# Autodesk Inventor assembly: Storage System Assembly
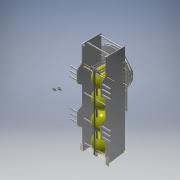
[picture p0: Inventor's stored thumbnail of the model, 180x180]
Saved by Autodesk Inventor 2019.4 (Build 234330000, 330)
## iProperties
Created: 2020-01-24
Part Number: Storage System Assembly
Document SubType Name: Assembly
Designer: admin
Mass: 6812.94 g
Surface Area: 16983.8 cm^2
Volume: 14320.1 cm^3
Density: 0.47576 g/cm^3
Author: admin
## Documents named in this file (18)
- C:\Users\admin\Desktop\FRC 2020 Engineering\GitHub\7738-2020\Robot V2\Storage System\Storage System Assembly.iam
- C:\Users\admin\Desktop\FRC 2020 Engineering\GitHub\7738-2020\Robot V2\Storage System\Storage Side Plate.ipt
- C:\Users\admin\Desktop\FRC 2020 Engineering\GitHub\7738-2020\Robot V2\Storage System\Storage System Assembly\Design Accelerator\Synchronous Belts Transmission1.iam
- C:\Users\admin\Desktop\FRC 2020 Engineering\GitHub\7738-2020\Robot V2\Storage System\Storage System Assembly\Design Accelerator\Synchronous Belts Transmission3.iam
- C:\Users\admin\Desktop\FRC 2020 Engineering\GitHub\7738-2020\Robot V2\Storage System\Storage System Assembly\Design Accelerator\Synchronous Belts Transmission4.iam
- C:\Users\admin\Desktop\FRC 2020 Engineering\GitHub\7738-2020\Robot V2\Storage System\Storage System Assembly\Design Accelerator\Synchronous Belts Transmission5.iam
- C:\Users\admin\Desktop\FRC 2020 Engineering\GitHub\7738-2020\Robot V2\Storage System\Storage System Assembly\Design Accelerator\Synchronous Belts Transmission6.iam
- C:\Users\admin\Desktop\FRC 2020 Engineering\GitHub\7738-2020\Power Cell.ipt
- C:\Users\admin\Desktop\FRC 2020 Engineering\GitHub\7738-2020\Robot V2\Turret\F6800.ipt
- C:\Users\admin\Desktop\FRC 2020 Engineering\GitHub\7738-2020\Robot V2\Storage System\Turret Support 2.ipt
- C:\Users\admin\Desktop\FRC 2020 Engineering\GitHub\7738-2020\Robot V2\Storage System\Turret Support.ipt
- C:\Users\admin\Desktop\FRC 2020 Engineering\GitHub\7738-2020\Robot V2\Storage System\Mounting Bracket.ipt
- C:\Users\admin\Desktop\FRC 2020 Engineering\GitHub\7738-2020\Robot V2\Storage System\Mounting Bracket 2.ipt
- C:\Users\admin\Desktop\FRC 2020 Engineering\GitHub\7738-2020\Robot V2\Storage System\Storage Plate Spacer.ipt
- C:\Users\admin\Desktop\FRC 2020 Engineering\GitHub\7738-2020\Robot V2\Storage System\Turret Bracket.ipt
- C:\Users\admin\Desktop\FRC 2020 Engineering\GitHub\7738-2020\Robot V2\Storage System\Small Support.ipt
- C:\Users\admin\Desktop\FRC 2020 Engineering\GitHub\7738-2020\Robot V2\Turret\Storage mounting spacers.ipt
- C:\Users\admin\Desktop\FRC 2020 Engineering\GitHub\7738-2020\Upper Stage\KFL08.ipt
## Components (61 placed, 13 different names)
1. Storage Side Plate:1 — Mate:1, Mate:3, Flush:2, Mate:14, Mate:15, Mate:16, Mate:17, Mate:25, Mate:26, Mate:27, Mate:28, Mate:31, Mate:32, Mate:38, Flush:3, Mate:43, Flush:7, Flush:8, Mate:44, Mate:45, Mate:46, Mate:47, Mate:48, Mate:49, Mate:50, Mate:51, Mate:52, Mate:63, Flush:13, Flush:15, Mate:92, Flush:17, Mate:94, Mate:108, Mate:109, Mate:110, Mate:111, Mate:112, Mate:113, Mate:114, Mate:115, Mate:116, Mate:117, Mate:118, Mate:119
2. Storage Side Plate:2 — Mate:1, Flush:1, Mate:12, Mate:13, Mate:18, Mate:19, Mate:20, Mate:22, Mate:23, Mate:24, Mate:29, Mate:30, Mate:40, Flush:4, Mate:42, Flush:5, Flush:6, Mate:53, Mate:54, Mate:55, Mate:56, Mate:57, Mate:58, Mate:59, Mate:60, Mate:61, Flush:9, Mate:65, Flush:11, Mate:80, Flush:14, Mate:126, Mate:127, Mate:128, Mate:129, Mate:130, Mate:131, Mate:132, Mate:133, Mate:134, Mate:135, Mate:136, Mate:137
3. Synchronous Belts Transmission:1 [sub-assembly]
4. Synchronous Belts Transmission:2 [sub-assembly]
5. Synchronous Belts Transmission:3 [sub-assembly]
6. Synchronous Belts Transmission:4 [sub-assembly]
7. Synchronous Belts Transmission:5 [sub-assembly]
8. Power Cell:1 — Mate:4, Mate:8
9. Power Cell:2 — Mate:5, Mate:11
10. Power Cell:3 — Mate:6, Mate:9
11. Power Cell:4 — Mate:7, Mate:10
12. F6800:1 — Mate:13, Mate:24
13. F6800:2 — Mate:30
14. F6800:3 — Mate:19, Mate:22
15. F6800:4 — Mate:14, Mate:25
16. F6800:5 — Mate:15, Mate:26
17. F6800:7 — Mate:16, Mate:28
18. F6800:8 — Mate:17, Mate:27
19. F6800:9 — Mate:18, Mate:29
20. F6800:10 — Mate:20, Mate:23
21. F6800:11 — Mate:31, Mate:32
22. Mounting Bracket:1 — Mate:38, Flush:3, Flush:13
23. Mounting Bracket:2 — Mate:40, Flush:4, Flush:14
24. Mounting Bracket 2:1 — Mate:42, Flush:5, Flush:6
25. Mounting Bracket 2:2 — Mate:43, Flush:7, Flush:8
26. Storage Plate Spacer:1 — Mate:46, Mate:60
27. Storage Plate Spacer:2 — Mate:48, Mate:55
28. Storage Plate Spacer:3 — Mate:44, Mate:59
29. Storage Plate Spacer:4 — Mate:51, Mate:54
30. Storage Plate Spacer:5 — Mate:47, Mate:80
31. Storage Plate Spacer:6 — Mate:50, Mate:57
32. Storage Plate Spacer:7 — Mate:49, Mate:56
33. Storage Plate Spacer:8 — Mate:52, Mate:53
34. Storage Plate Spacer:9 — Mate:45, Mate:58
35. Turret Bracket:2 — Mate:61, Flush:9, Flush:11
36. Turret Bracket:3 — Mate:65, Flush:16
37. Turret Bracket:4 — Mate:63, Flush:15, Flush:16, Mate:95
38. Small Support:1 — Mate:104, Mate:107
39. Small Support:2 — Mate:102, Mate:103
40. Small Support:3 — Mate:105, Mate:106
41. Small Support:4 — Mate:99, Mate:100, Mate:101
42. Turret Bracket:5 — Mate:92, Flush:17, Mate:98, Mate:100, Mate:103
43. Turret Support 2:2 — Mate:97, Mate:98, Mate:99, Mate:101, Mate:102, Mate:104, Mate:105, Mate:106, Mate:107
44. Turret Support:3 — Mate:93, Mate:94, Mate:95, Mate:96, Mate:97
45. Storage mounting spacers:1 — Mate:108, Mate:119
46. Storage mounting spacers:2 — Mate:109, Mate:118
47. Storage mounting spacers:3 — Mate:110, Mate:117
48. Storage mounting spacers:4 — Mate:111, Mate:114
49. Storage mounting spacers:5 — Mate:112, Mate:115
50. Storage mounting spacers:6 — Mate:113, Mate:116
51. Storage mounting spacers:7 — Mate:126, Mate:137
52. Storage mounting spacers:8 — Mate:127, Mate:136
53. Storage mounting spacers:9 — Mate:128, Mate:135
54. Storage mounting spacers:10 — Mate:130, Mate:133
55. Storage mounting spacers:11 — Mate:129, Mate:134
56. Storage mounting spacers:12 — Mate:131, Mate:132
57. KFL08:1
58. KFL08:2
59. KFL08:3
60. KFL08:4
61. KFL08:5
## Relationships (110: Mate 95, Flush 15)
- Mate:1: Storage Side Plate:1 ↔ Storage Side Plate:2
- Mate:3 (114.3 mm): Storage Side Plate:1
- Flush:1 (114.3 mm): Storage Side Plate:2
- Mate:4: Power Cell:1
- Mate:5: Power Cell:2
- Mate:6: Power Cell:3
- Mate:7: Power Cell:4
- Mate:8: Power Cell:1
- Mate:9: Power Cell:3
- Mate:10: Power Cell:4
- Mate:11: Power Cell:2
- Mate:12: Storage Side Plate:2
- Flush:2: Storage Side Plate:1
- Mate:13: Storage Side Plate:2 ↔ F6800:1
- Mate:14: Storage Side Plate:1 ↔ F6800:4
- Mate:15: Storage Side Plate:1 ↔ F6800:5
- Mate:16: Storage Side Plate:1 ↔ F6800:7
- Mate:17: Storage Side Plate:1 ↔ F6800:8
- Mate:18: Storage Side Plate:2 ↔ F6800:9
- Mate:19: Storage Side Plate:2 ↔ F6800:3
- Mate:20: Storage Side Plate:2 ↔ F6800:10
- Mate:22 (0.2 mm): Storage Side Plate:2 ↔ F6800:3
- Mate:23 (0.2 mm): Storage Side Plate:2 ↔ F6800:10
- Mate:24 (0.2 mm): Storage Side Plate:2 ↔ F6800:1
- Mate:25 (0.2 mm): Storage Side Plate:1 ↔ F6800:4
- Mate:26 (0.2 mm): Storage Side Plate:1 ↔ F6800:5
- Mate:27 (0.2 mm): Storage Side Plate:1 ↔ F6800:8
- Mate:28 (0.2 mm): Storage Side Plate:1 ↔ F6800:7
- Mate:29 (0.2 mm): Storage Side Plate:2 ↔ F6800:9
- Mate:30 (0.2 mm): Storage Side Plate:2 ↔ F6800:2
- Mate:31: Storage Side Plate:1 ↔ F6800:11
- Mate:32 (0.2 mm): Storage Side Plate:1 ↔ F6800:11
- Mate:38: Storage Side Plate:1 ↔ Mounting Bracket:1
- Flush:3 (5 mm): Storage Side Plate:1 ↔ Mounting Bracket:1
- Mate:40: Storage Side Plate:2 ↔ Mounting Bracket:2
- Flush:4 (5 mm): Storage Side Plate:2 ↔ Mounting Bracket:2
- Mate:42: Storage Side Plate:2 ↔ Mounting Bracket 2:1
- Mate:43: Storage Side Plate:1 ↔ Mounting Bracket 2:2
- Flush:5: Storage Side Plate:2 ↔ Mounting Bracket 2:1
- Flush:6: Storage Side Plate:2 ↔ Mounting Bracket 2:1
- Flush:7: Storage Side Plate:1 ↔ Mounting Bracket 2:2
- Flush:8: Storage Side Plate:1 ↔ Mounting Bracket 2:2
- Mate:44: Storage Side Plate:1 ↔ Storage Plate Spacer:3
- Mate:45: Storage Side Plate:1 ↔ Storage Plate Spacer:9
- Mate:46: Storage Side Plate:1 ↔ Storage Plate Spacer:1
- Mate:47: Storage Side Plate:1 ↔ Storage Plate Spacer:5
- Mate:48: Storage Side Plate:1 ↔ Storage Plate Spacer:2
- Mate:49: Storage Side Plate:1 ↔ Storage Plate Spacer:7
- Mate:50: Storage Side Plate:1 ↔ Storage Plate Spacer:6
- Mate:51: Storage Side Plate:1 ↔ Storage Plate Spacer:4
- Mate:52: Storage Side Plate:1 ↔ Storage Plate Spacer:8
- Mate:53: Storage Side Plate:2 ↔ Storage Plate Spacer:8
- Mate:54: Storage Side Plate:2 ↔ Storage Plate Spacer:4
- Mate:55: Storage Side Plate:2 ↔ Storage Plate Spacer:2
- Mate:56: Storage Side Plate:2 ↔ Storage Plate Spacer:7
- Mate:57: Storage Side Plate:2 ↔ Storage Plate Spacer:6
- Mate:58: Storage Side Plate:2 ↔ Storage Plate Spacer:9
- Mate:59: Storage Side Plate:2 ↔ Storage Plate Spacer:3
- Mate:60: Storage Side Plate:2 ↔ Storage Plate Spacer:1
- Mate:61: Storage Side Plate:2 ↔ Turret Bracket:2
- Flush:9: Storage Side Plate:2 ↔ Turret Bracket:2
- Mate:63: Storage Side Plate:1 ↔ Turret Bracket:4
- Mate:65: Storage Side Plate:2 ↔ Turret Bracket:3
- Flush:11 (400 mm): Storage Side Plate:2 ↔ Turret Bracket:2
- Mate:80: Storage Side Plate:2 ↔ Storage Plate Spacer:5
- Flush:13: Storage Side Plate:1 ↔ Mounting Bracket:1
- Flush:14: Storage Side Plate:2 ↔ Mounting Bracket:2
- Flush:15: Storage Side Plate:1 ↔ Turret Bracket:4
- Flush:16: Turret Bracket:3 ↔ Turret Bracket:4
- Mate:92: Storage Side Plate:1 ↔ Turret Bracket:5
- Flush:17: Storage Side Plate:1 ↔ Turret Bracket:5
- Mate:93: Turret Support:3
- Mate:94: Storage Side Plate:1 ↔ Turret Support:3
- Mate:95: Turret Bracket:4 ↔ Turret Support:3
- Mate:96: Turret Support:3
- Mate:97: Turret Support 2:2 ↔ Turret Support:3
- Mate:98: Turret Bracket:5 ↔ Turret Support 2:2
- Mate:99: Small Support:4 ↔ Turret Support 2:2
- Mate:100: Small Support:4 ↔ Turret Bracket:5
- Mate:101: Small Support:4 ↔ Turret Support 2:2
- Mate:102: Small Support:2 ↔ Turret Support 2:2
- Mate:103: Small Support:2 ↔ Turret Bracket:5
- Mate:104: Small Support:1 ↔ Turret Support 2:2
- Mate:105: Small Support:3 ↔ Turret Support 2:2
- Mate:106: Small Support:3 ↔ Turret Support 2:2
- Mate:107: Small Support:1 ↔ Turret Support 2:2
- Mate:108: Storage Side Plate:1 ↔ Storage mounting spacers:1
- Mate:109: Storage Side Plate:1 ↔ Storage mounting spacers:2
- Mate:110: Storage Side Plate:1 ↔ Storage mounting spacers:3
- Mate:111: Storage Side Plate:1 ↔ Storage mounting spacers:4
- Mate:112: Storage Side Plate:1 ↔ Storage mounting spacers:5
- Mate:113: Storage Side Plate:1 ↔ Storage mounting spacers:6
- Mate:114: Storage Side Plate:1 ↔ Storage mounting spacers:4
- Mate:115: Storage Side Plate:1 ↔ Storage mounting spacers:5
- Mate:116: Storage Side Plate:1 ↔ Storage mounting spacers:6
- Mate:117: Storage Side Plate:1 ↔ Storage mounting spacers:3
- Mate:118: Storage Side Plate:1 ↔ Storage mounting spacers:2
- Mate:119: Storage Side Plate:1 ↔ Storage mounting spacers:1
- Mate:126: Storage Side Plate:2 ↔ Storage mounting spacers:7
- Mate:127: Storage Side Plate:2 ↔ Storage mounting spacers:8
- Mate:128: Storage Side Plate:2 ↔ Storage mounting spacers:9
- Mate:129: Storage Side Plate:2 ↔ Storage mounting spacers:11
- Mate:130: Storage Side Plate:2 ↔ Storage mounting spacers:10
- Mate:131: Storage Side Plate:2 ↔ Storage mounting spacers:12
- Mate:132: Storage Side Plate:2 ↔ Storage mounting spacers:12
- Mate:133: Storage Side Plate:2 ↔ Storage mounting spacers:10
- Mate:134: Storage Side Plate:2 ↔ Storage mounting spacers:11
- Mate:135: Storage Side Plate:2 ↔ Storage mounting spacers:9
- Mate:136: Storage Side Plate:2 ↔ Storage mounting spacers:8
- Mate:137: Storage Side Plate:2 ↔ Storage mounting spacers:7
